# Autodesk Inventor assembly: FRAME
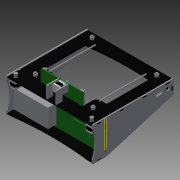
[picture p0: Inventor's stored thumbnail of the model, 180x180]
Saved by Autodesk Inventor 2013 (Build 170138000, 138)
## iProperties
Created: 2014-03-03
Part Number: FRAME
Document SubType Name: Assembly
Designer: employee
Author: employee
## Documents named in this file (18)
- C:\Users\employee\Desktop\CoreXZ\FRAME.iam
- C:\Users\employee\Desktop\CoreXZ\FRAME.ipt
- C:\Users\employee\Desktop\CoreXZ\M8X290 ROD.ipt
- C:\Users\employee\Desktop\CoreXZ\M8 WASHER.ipt
- C:\Users\employee\Desktop\CoreXZ\608.ipt
- C:\Users\employee\Desktop\CoreXZ\M8X30.ipt
- C:\Users\employee\Desktop\CoreXZ\M8 NUT.ipt
- C:\Users\employee\Desktop\CoreXZ\FRAME BOTTOM.ipt
- C:\Users\employee\Desktop\CoreXZ\Y BEARING BLOCK.ipt
- C:\Users\employee\Desktop\CoreXZ\LM8UU.ipt
- C:\Users\employee\Desktop\CoreXZ\STEPPER.ipt
- C:\Users\employee\Desktop\CoreXZ\STEPPER OFFSET.ipt
- C:\Users\employee\Desktop\CoreXZ\SPOOL.ipt
- C:\Users\employee\Desktop\CoreXZ\FRAME SIDE.ipt
- C:\Users\employee\Desktop\CoreXZ\POWER SUPPLY.ipt
- C:\Users\employee\Desktop\CoreXZ\STRUT.ipt
- C:\Users\employee\Desktop\CoreXZ\OVERHANG SUPPORT.ipt
- C:\Users\employee\Desktop\CoreXZ\ELECTRONICS.ipt
## Components (47 placed, 17 different names)
1. FRAME:1 — Insert:1, Insert:2, Insert:3, Insert:4, Insert:11, Insert:12, Mate:1, Mate:2, Flush:1, Insert:20, Insert:21, Insert:26, Insert:27, Insert:30, Insert:31, Angle:3, Angle:4, Angle:5, Angle:6, Mate:6, Flush:8, Mate:10, Mate:12, Mate:14
2. M8X290 ROD:1 — Insert:1
3. M8X290 ROD:2 — Insert:2
4. M8 WASHER:1 — Insert:3, Insert:5
5. M8 WASHER:2 — Insert:4, Insert:7
6. 608:1 — Insert:5, Insert:6
7. 608:2 — Insert:6, Insert:9
8. 608:3 — Insert:7, Insert:8
9. 608:4 — Insert:8, Insert:10
10. M8X30:1 — Insert:9
11. M8X30:2 — Insert:10
12. M8 NUT:1 — Insert:11
13. M8 NUT:2 — Insert:12
14. FRAME BOTTOM:1 — Mate:1, Mate:2, Flush:1, Mate:3, Mate:4, Flush:2, Flush:3, Flush:4, Flush:5, Insert:17, Angle:1, Angle:2, Flush:6, Flush:7, Mate:5, Mate:7, Flush:11, Mate:11, Mate:13, Mate:17
15. Y BEARING BLOCK:1 — Mate:3, Flush:4, Flush:5, Insert:15, Insert:16
16. Y BEARING BLOCK:2 — Mate:4, Flush:2, Flush:3, Insert:13, Insert:14
17. LM8UU:1 — Insert:13
18. LM8UU:2 — Insert:14
19. LM8UU:3 — Insert:16
20. LM8UU:4 — Insert:15
21. STEPPER:1 — Insert:18, Angle:2, Insert:19
22. STEPPER OFFSET:1 — Insert:17, Angle:1, Insert:18, Mate:15, Mate:16
23. SPOOL:1 — Insert:19
24. M8 WASHER:3 — Insert:20, Insert:22
25. M8 WASHER:4 — Insert:21, Insert:24
26. 608:5 — Insert:22, Insert:23
27. 608:6 — Insert:23, Insert:29
28. 608:7 — Insert:24, Insert:25
29. 608:8 — Insert:25, Insert:28
30. M8 NUT:3 — Insert:26
31. M8 NUT:4 — Insert:27
32. M8X30:3 — Insert:29
33. M8X30:4 — Insert:28
34. STEPPER OFFSET:2 — Insert:30, Angle:4, Insert:32
35. STEPPER OFFSET:3 — Insert:31, Angle:3, Insert:33
36. STEPPER:2 — Insert:33, Angle:5, Insert:34
37. STEPPER:3 — Insert:32, Angle:6, Insert:35
38. SPOOL:2 — Insert:34
39. SPOOL:3 — Insert:35
40. FRAME SIDE:1 — Flush:6, Flush:7, Mate:8, Mate:9, Flush:9, Flush:10
41. POWER SUPPLY:1 — Mate:5
42. STRUT:1 — Mate:7, Mate:8, Flush:11
43. STRUT:2 — Mate:6, Mate:9, Flush:8
44. FRAME SIDE:2 — Mate:10, Flush:9, Flush:10
45. OVERHANG SUPPORT:1 — Mate:11, Mate:12, Mate:16
46. OVERHANG SUPPORT:2 — Mate:13, Mate:14, Mate:15
47. ELECTRONICS:1 — Mate:17
## Relationships (69: Insert 35, Mate 17, Flush 11, Angle 6)
- Insert:1: FRAME:1 ↔ M8X290 ROD:1
- Insert:2: FRAME:1 ↔ M8X290 ROD:2
- Insert:3: FRAME:1 ↔ M8 WASHER:1
- Insert:4: FRAME:1 ↔ M8 WASHER:2
- Insert:5: M8 WASHER:1 ↔ 608:1
- Insert:6: 608:1 ↔ 608:2
- Insert:7: M8 WASHER:2 ↔ 608:3
- Insert:8: 608:3 ↔ 608:4
- Insert:9: 608:2 ↔ M8X30:1
- Insert:10: 608:4 ↔ M8X30:2
- Insert:11: FRAME:1 ↔ M8 NUT:1
- Insert:12: FRAME:1 ↔ M8 NUT:2
- Mate:1: FRAME:1 ↔ FRAME BOTTOM:1
- Mate:2: FRAME:1 ↔ FRAME BOTTOM:1
- Flush:1: FRAME:1 ↔ FRAME BOTTOM:1
- Mate:3: FRAME BOTTOM:1 ↔ Y BEARING BLOCK:1
- Mate:4: FRAME BOTTOM:1 ↔ Y BEARING BLOCK:2
- Flush:2: FRAME BOTTOM:1 ↔ Y BEARING BLOCK:2
- Flush:3: FRAME BOTTOM:1 ↔ Y BEARING BLOCK:2
- Flush:4: FRAME BOTTOM:1 ↔ Y BEARING BLOCK:1
- Flush:5: FRAME BOTTOM:1 ↔ Y BEARING BLOCK:1
- Insert:13: Y BEARING BLOCK:2 ↔ LM8UU:1
- Insert:14: Y BEARING BLOCK:2 ↔ LM8UU:2
- Insert:15: Y BEARING BLOCK:1 ↔ LM8UU:4
- Insert:16: Y BEARING BLOCK:1 ↔ LM8UU:3
- Insert:17: FRAME BOTTOM:1 ↔ STEPPER OFFSET:1
- Angle:1 (0 deg): FRAME BOTTOM:1 ↔ STEPPER OFFSET:1
- Insert:18: STEPPER:1 ↔ STEPPER OFFSET:1
- Angle:2 (0 deg): FRAME BOTTOM:1 ↔ STEPPER:1
- Insert:19 (-1 mm): STEPPER:1 ↔ SPOOL:1
- Insert:20: FRAME:1 ↔ M8 WASHER:3
- Insert:21: FRAME:1 ↔ M8 WASHER:4
- Insert:22: M8 WASHER:3 ↔ 608:5
- Insert:23: 608:5 ↔ 608:6
- Insert:24: M8 WASHER:4 ↔ 608:7
- Insert:25: 608:7 ↔ 608:8
- Insert:26: FRAME:1 ↔ M8 NUT:3
- Insert:27: FRAME:1 ↔ M8 NUT:4
- Insert:28: 608:8 ↔ M8X30:4
- Insert:29: 608:6 ↔ M8X30:3
- Insert:30: FRAME:1 ↔ STEPPER OFFSET:2
- Insert:31: FRAME:1 ↔ STEPPER OFFSET:3
- Angle:3 (0 deg): FRAME:1 ↔ STEPPER OFFSET:3
- Angle:4 (0 deg): FRAME:1 ↔ STEPPER OFFSET:2
- Insert:32: STEPPER OFFSET:2 ↔ STEPPER:3
- Insert:33: STEPPER OFFSET:3 ↔ STEPPER:2
- Angle:5 (0 deg): FRAME:1 ↔ STEPPER:2
- Angle:6 (0 deg): FRAME:1 ↔ STEPPER:3
- Insert:34 (-2 mm): STEPPER:2 ↔ SPOOL:2
- Insert:35 (-2 mm): STEPPER:3 ↔ SPOOL:3
- Flush:6: FRAME BOTTOM:1 ↔ FRAME SIDE:1
- Flush:7: FRAME BOTTOM:1 ↔ FRAME SIDE:1
- Mate:5: FRAME BOTTOM:1 ↔ POWER SUPPLY:1
- Mate:6: FRAME:1 ↔ STRUT:2
- Mate:7: FRAME BOTTOM:1 ↔ STRUT:1
- Mate:8: FRAME SIDE:1 ↔ STRUT:1
- Mate:9: FRAME SIDE:1 ↔ STRUT:2
- Flush:8 (5 mm): FRAME:1 ↔ STRUT:2
- Mate:10: FRAME:1 ↔ FRAME SIDE:2
- Flush:9: FRAME SIDE:1 ↔ FRAME SIDE:2
- Flush:10: FRAME SIDE:1 ↔ FRAME SIDE:2
- Flush:11 (5 mm): FRAME BOTTOM:1 ↔ STRUT:1
- Mate:11: FRAME BOTTOM:1 ↔ OVERHANG SUPPORT:1
- Mate:12: FRAME:1 ↔ OVERHANG SUPPORT:1
- Mate:13: FRAME BOTTOM:1 ↔ OVERHANG SUPPORT:2
- Mate:14: FRAME:1 ↔ OVERHANG SUPPORT:2
- Mate:15 (5 mm): STEPPER OFFSET:1 ↔ OVERHANG SUPPORT:2
- Mate:16 (5 mm): STEPPER OFFSET:1 ↔ OVERHANG SUPPORT:1
- Mate:17: FRAME BOTTOM:1 ↔ ELECTRONICS:1
